# Autodesk Inventor assembly: Supporto saldato pistone 2 - Trasporto
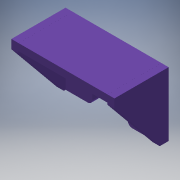
[picture p0: Inventor's stored thumbnail of the model, 180x180]
Saved by Autodesk Inventor 2018 (Build 220112000, 112)
## iProperties
Created: 2020-06-01
Part Number: Supporto saldato pistone 2 - Trasporto
Material: Generico
Document SubType Name: Weldment
Designer: Francesco
Weld Material: Welded Aluminum-6061
Author: Francesco
## Documents named in this file (4)
- C:\Users\Francesco\no-brim\Meccanica\Progetto Inventor no-brim\Assiemi\Supporto saldato pistone 2 - Trasporto.iam
- C:\Users\Francesco\no-brim\Meccanica\Progetto Inventor no-brim\Parti\Base supp.saldato.ipt
- C:\Users\Francesco\no-brim\Meccanica\Progetto Inventor no-brim\Parti\Fianchi supp.saldato.ipt
- C:\Users\Francesco\no-brim\Meccanica\Progetto Inventor no-brim\Parti\Appoggio pistone supp.saldato.ipt
## Components (5 placed, 3 different names)
1. Base supp.saldato:1 — Coincidente:1, Allineato:1, Allineato:2, Coincidente:2, Allineato:3, Allineato:4
2. Fianchi supp.saldato:1 — Coincidente:1, Allineato:1, Allineato:2, Allineato:7, Allineato:8, Coincidente:4
3. Fianchi supp.saldato:2 — Coincidente:2, Allineato:3, Allineato:4, Coincidente:5, Allineato:9, Allineato:10
4. Appoggio pistone supp.saldato:1 — Coincidente:5, Allineato:9, Allineato:10
5. Appoggio pistone supp.saldato:2 — Allineato:7, Allineato:8, Coincidente:4
## Relationships (12: Flush 8, Mate 4)
- Coincidente:1 [Mate]: Base supp.saldato:1 ↔ Fianchi supp.saldato:1
- Allineato:1 [Flush]: Base supp.saldato:1 ↔ Fianchi supp.saldato:1
- Allineato:2 [Flush]: Base supp.saldato:1 ↔ Fianchi supp.saldato:1
- Coincidente:2 [Mate]: Base supp.saldato:1 ↔ Fianchi supp.saldato:2
- Allineato:3 [Flush]: Base supp.saldato:1 ↔ Fianchi supp.saldato:2
- Allineato:4 [Flush]: Base supp.saldato:1 ↔ Fianchi supp.saldato:2
- Allineato:7 [Flush]: Fianchi supp.saldato:1 ↔ Appoggio pistone supp.saldato:2
- Allineato:8 [Flush]: Fianchi supp.saldato:1 ↔ Appoggio pistone supp.saldato:2
- Coincidente:4 [Mate]: Fianchi supp.saldato:1 ↔ Appoggio pistone supp.saldato:2
- Coincidente:5 [Mate]: Fianchi supp.saldato:2 ↔ Appoggio pistone supp.saldato:1
- Allineato:9 [Flush]: Fianchi supp.saldato:2 ↔ Appoggio pistone supp.saldato:1
- Allineato:10 [Flush]: Fianchi supp.saldato:2 ↔ Appoggio pistone supp.saldato:1
